# Autodesk Inventor assembly: ASSEMBLY
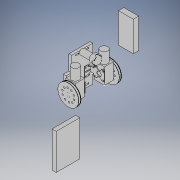
[picture p0: Inventor's stored thumbnail of the model, 180x180]
Saved by Autodesk Inventor 2016 (Build 200138000, 138)
## iProperties
Created: 2017-09-08
Part Number: ASSEMBLY
Document SubType Name: Assembly
Designer: Student
Author: Student
## Documents named in this file (9)
- F:\sumo bot\ASSEMBLY.iam
- F:\sumo bot\msheehan_frame_2.ipt
- F:\sumo bot\msheehan_motor_mount.ipt
- F:\sumo bot\msheehan_motor.ipt
- F:\sumo bot\msheehan_caster.ipt
- F:\sumo bot\msheehan_bearing.ipt
- F:\sumo bot\msheehan_small_breadboard.ipt
- F:\sumo bot\msheehan_wheel_small.ipt
- F:\sumo bot\msheehan_battery.ipt
## Components (11 placed, 8 different names)
1. msheehan_frame_2:1 — Rotational:1, Rotational:2, Rigid:3
2. msheehan_motor_mount:1 — Rotational:1, Rigid:2
3. msheehan_motor_mount:2 — Rotational:2, Rigid:4
4. msheehan_motor:1 — Rigid:2, Rotational:4
5. msheehan_caster:1 — Rigid:3, Ball:1
6. msheehan_bearing:1 — Ball:1
7. msheehan_small_breadboard:1
8. msheehan_motor:2 — Rigid:4, Rotational:3
9. msheehan_wheel_small:1 — Rotational:3
10. msheehan_wheel_small:2 — Rotational:4
11. msheehan_battery:1
## Relationships (8: RevoluteJoint 4, WeldJoint 3, BallJoint 1)
- Rotational:1 [RevoluteJoint]: msheehan_frame_2:1 ↔ msheehan_motor_mount:1
- Rotational:2 [RevoluteJoint]: msheehan_frame_2:1 ↔ msheehan_motor_mount:2
- Rigid:2 [WeldJoint]: msheehan_motor_mount:1 ↔ msheehan_motor:1
- Rigid:3 [WeldJoint]: msheehan_frame_2:1 ↔ msheehan_caster:1
- Rigid:4 [WeldJoint]: msheehan_motor_mount:2 ↔ msheehan_motor:2
- Ball:1: msheehan_caster:1 ↔ msheehan_bearing:1
- Rotational:3 [RevoluteJoint]: msheehan_motor:2 ↔ msheehan_wheel_small:1
- Rotational:4 [RevoluteJoint]: msheehan_motor:1 ↔ msheehan_wheel_small:2
